# Autodesk Inventor assembly: fast_z_axis
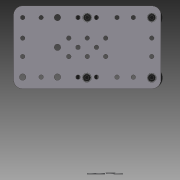
[picture p0: Inventor's stored thumbnail of the model, 180x180]
Saved by Autodesk Inventor 2013 (Build 170138000, 138)
## iProperties
Created: 2013-06-22
Part Number: fast_z_axis
Document SubType Name: Assembly
Designer: Brett
Author: Brett
## Documents named in this file (7)
- C:\Users\Brett\Documents\GitHub\BigOko\bb_assemblies\fast_z_axis.iam
- C:\Users\Brett\Documents\GitHub\BigOko\Parts\MSK01-01.ipt
- C:\Users\Brett\Documents\GitHub\BigOko\Parts\MSK01-04.ipt
- C:\Users\Brett\Documents\GitHub\BigOko\Parts\SM-H03.ipt
- C:\Users\Brett\Documents\GitHub\BigOko\Parts\MSK01-05A.ipt
- C:\Users\Brett\Documents\GitHub\BigOko\Parts\SM-H08.ipt
- C:\Users\Brett\Documents\GitHub\BigOko\Parts\SM-H04.ipt
## Components (31 placed, 6 different names)
1. MSK01-01:1 — Insert:1, Insert:2, Insert:3, Insert:4, Insert:9, Insert:10
2. MSK01-04:1 — Insert:2, Insert:6, Insert:24
3. MSK01-04:2 — Insert:1, Insert:5, Insert:23
4. SM-H03:1 — Insert:3, Insert:21
5. SM-H03:2 — Insert:6, Insert:27
6. SM-H03:3 — Insert:30, Insert:32
7. SM-H03:4
8. SM-H03:5
9. SM-H03:6 — Insert:26, Insert:28
10. SM-H03:7 — Insert:10, Insert:14
11. SM-H03:8 — Insert:4, Insert:22
12. SM-H03:9 — Insert:24, Insert:25
13. SM-H03:10 — Insert:9, Insert:13
14. SM-H03:11 — Insert:17, Insert:33
15. SM-H03:12
16. SM-H03:13
17. SM-H03:14 — Insert:18, Insert:34
18. SM-H03:15 — Insert:23, Insert:29
19. SM-H03:16 — Insert:5, Insert:31
20. MSK01-05A:1 — Insert:29, Insert:30
21. MSK01-05A:2 — Insert:25, Insert:26
22. MSK01-05A:3 — Insert:13, Insert:17
23. MSK01-05A:4 — Insert:14, Insert:18
24. SM-H08:1 — Insert:31
25. SM-H08:2 — Insert:27
26. SM-H08:3 — Insert:21
27. SM-H08:4 — Insert:22
28. SM-H04:1 — Insert:34
29. SM-H04:2 — Insert:33
30. SM-H04:3 — Insert:32
31. SM-H04:4 — Insert:28
## Relationships (26: Insert 26)
- Insert:1: MSK01-01:1 ↔ MSK01-04:2
- Insert:2: MSK01-01:1 ↔ MSK01-04:1
- Insert:3: MSK01-01:1 ↔ SM-H03:1
- Insert:4: MSK01-01:1 ↔ SM-H03:8
- Insert:5: MSK01-04:2 ↔ SM-H03:16
- Insert:6: MSK01-04:1 ↔ SM-H03:2
- Insert:9: MSK01-01:1 ↔ SM-H03:10
- Insert:10: MSK01-01:1 ↔ SM-H03:7
- Insert:13: SM-H03:10 ↔ MSK01-05A:3
- Insert:14: SM-H03:7 ↔ MSK01-05A:4
- Insert:17: SM-H03:11 ↔ MSK01-05A:3
- Insert:18: SM-H03:14 ↔ MSK01-05A:4
- Insert:21: SM-H03:1 ↔ SM-H08:3
- Insert:22: SM-H03:8 ↔ SM-H08:4
- Insert:23 (1.905 mm): MSK01-04:2 ↔ SM-H03:15
- Insert:24 (1.905 mm): MSK01-04:1 ↔ SM-H03:9
- Insert:25: SM-H03:9 ↔ MSK01-05A:2
- Insert:26: SM-H03:6 ↔ MSK01-05A:2
- Insert:27: SM-H03:2 ↔ SM-H08:2
- Insert:28: SM-H03:6 ↔ SM-H04:4
- Insert:29: SM-H03:15 ↔ MSK01-05A:1
- Insert:30: SM-H03:3 ↔ MSK01-05A:1
- Insert:31: SM-H03:16 ↔ SM-H08:1
- Insert:32: SM-H03:3 ↔ SM-H04:3
- Insert:33: SM-H03:11 ↔ SM-H04:2
- Insert:34: SM-H03:14 ↔ SM-H04:1
